(part 1 of 2)
# Autodesk Inventor assembly: #Spindexer
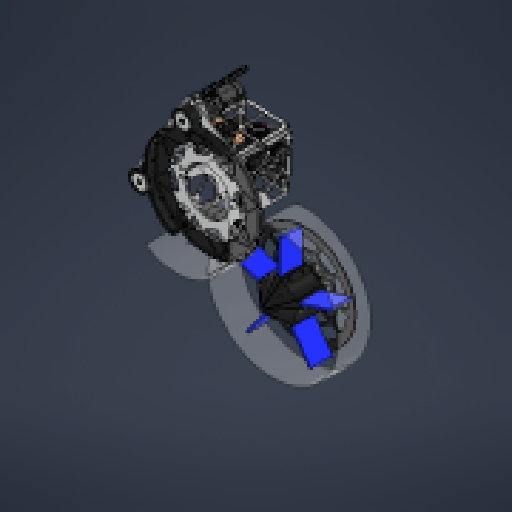
[picture p0: Inventor's stored thumbnail of the model, 512x512]
Saved by Autodesk Inventor 2026.1 (Build 301233020, 233B)
## iProperties
Created: 2026-02-05
Part Number: #Spindexer
Document SubType Name: Assembly
Designer: Owen L
Mass: 7699.55 g
Surface Area: 21817.8 cm^2
Volume: 5845.98 cm^3
Density: 1.31707 g/cm^3
Author: Owen L
## Documents named in this file (69)
- C:\Users\Owen\Documents\GitHub\2026-Robot-Mechanical\Spindexer\#Spindexer.iam
- C:\Users\Owen\Documents\GitHub\2026-Robot-Mechanical\Spindexer\3DPRINT,HUB.ipt
- C:\Users\Owen\Documents\GitHub\2026-Robot-Mechanical\Spindexer\3DPRINT,HUB,CONE.ipt
- C:\Users\Owen\Documents\GitHub\2026-Robot-Mechanical\Spindexer\PLATE,WALL.ipt
- C:\Users\Owen\Documents\GitHub\2026-Robot-Mechanical\Spindexer\PLATE,BOTTOM.ipt
- C:\Users\Owen\Documents\GitHub\2026-Robot-Mechanical\Spindexer\STOCK,HEX,SHAFT,HUB.ipt
- C:\Users\Owen\Documents\GitHub\2026-Robot-Mechanical\Spindexer\PLATE,KICKER,OUTSIDE.ipt
- C:\Users\Owen\Documents\GitHub\2026-Robot-Mechanical\Spindexer\3DPRINT,KICKER,RAMP.ipt
- C:\Users\Owen\Documents\GitHub\2026-Robot-Mechanical\Spindexer\PLATE,KICKER,INSIDE.ipt
- C:\Users\Owen\Documents\GitHub\2026-Robot-Mechanical\Spindexer\STOCK,HEX,SHAFT,KICKER,FRONT.ipt
- C:\Users\Owen\Documents\GitHub\2026-Robot-Mechanical\Spindexer\STOCK,HEX,SHAFT,KICKER,BACK.ipt
- C:\Users\Owen\Documents\GitHub\2026-Robot-Mechanical\#1_CAD Library\Power Transmission\Bearings\PURCHASED,HEX_BEARING.ipt
- C:\Users\Owen\Documents\GitHub\2026-Robot-Mechanical\#1_CAD Library\Power Transmission\VersaPlanetary\GEARBOX,VERSAPLANETARY,SINGLE-STAGE,HEX-SHAFT,0.5IN.ipt
- C:\Users\Owen\Documents\GitHub\2026-Robot-Mechanical\#1_CAD Library\Power Transmission\VersaPlanetary\ADAPTER,CIM-NEO,VERSAPLANETARY.ipt
- C:\Users\Owen\Documents\GitHub\2026-Robot-Mechanical\#1_CAD Library\Motors\MOTOR,REV,NEO,V1-1.ipt
- C:\Users\Owen\Documents\GitHub\2026-Robot-Mechanical\Spindexer\PLATE,NUT-BLOCK,3-LONG.ipt
- C:\Users\Owen\Documents\GitHub\2026-Robot-Mechanical\Spindexer\PLATE,NUT-BLOCK,2-LONG.ipt
- C:\Users\Owen\Documents\GitHub\2026-Robot-Mechanical\Spindexer\PLATE,NUT-BLOCK,1-LONG.ipt
- C:\Users\Owen\Documents\GitHub\2026-Robot-Mechanical\#1_CAD Library\Electronics\CONTROLS,SPARK_MAX.ipt
- C:\Users\Owen\Documents\GitHub\2026-Robot-Mechanical\Spindexer\3DPRINT,SPARK_MAX,MOUNT.ipt
- C:\Users\Owen\Documents\GitHub\2026-Robot-Mechanical\Spindexer\PLATE,KICKER,BACK.ipt
- C:\Users\Owen\Documents\GitHub\2026-Robot-Mechanical\Spindexer\PLATE,NUT-BLOCK,L-SHAPE.ipt
- C:\Users\Owen\Documents\GitHub\2026-Robot-Mechanical\Spindexer\STANDIN,BELT,70T,HTD5mm.ipt
- C:\Users\Owen\Documents\GitHub\2026-Robot-Mechanical\Spindexer\STANDIN,BELT,85T,HTD5mm.ipt
- C:\Users\Owen\Documents\GitHub\2026-Robot-Mechanical\#1_CAD Library\Building Materials\Fasteners\Bolts\PURCHASED,10-32x0.5in,BUTTONHEAD,BOLT.ipt
- C:\Users\Owen\Documents\GitHub\2026-Robot-Mechanical\#1_CAD Library\Building Materials\Fasteners\Nuts\PURCHASED,NYLOCK,10-32,NUT.ipt
- C:\Users\Owen\Documents\GitHub\2026-Robot-Mechanical\#1_CAD Library\Building Materials\Fasteners\Bolts\PURCHASED,10-32x0.625in,BUTTONHEAD,BOLT.ipt
- C:\Users\Owen\Documents\GitHub\2026-Robot-Mechanical\Spindexer\PLATE,NUT-BLOCK,SINGLE-L.ipt
- C:\Users\Owen\Documents\GitHub\2026-Robot-Mechanical\Spindexer\PLATE,SHOOTER,MOUNT.ipt
- C:\Users\Owen\Documents\GitHub\2026-Robot-Mechanical\Spindexer\PLATE,TURRET,ENCODER,GEAR.ipt
- C:\Users\Owen\Documents\GitHub\2026-Robot-Mechanical\Spindexer\PLATE,TURRET,PINNION,GEAR.ipt
- C:\Users\Owen\Documents\GitHub\2026-Robot-Mechanical\Spindexer\PLATE,TURRET,MOTOR,MOUNT.ipt
- C:\Users\Owen\Documents\GitHub\2026-Robot-Mechanical\#1_CAD Library\Electronics\CONTROLS,ENCODER,HEX_BORE.ipt
- C:\Users\Owen\Documents\GitHub\2026-Robot-Mechanical\Spindexer\STOCK,HEX,SHAFT,TURRET,DRIVE.ipt
- C:\Users\Owen\Documents\GitHub\2026-Robot-Mechanical\Spindexer\STOCK,HEX,SHAFT,TURRET,ENCODER.ipt
- C:\Users\Owen\Documents\GitHub\2026-Robot-Mechanical\Spindexer\3DPRINT,TURRET,HEX,SPACER.ipt
- C:\Users\Owen\Documents\GitHub\2026-Robot-Mechanical\Spindexer\STOCK,CHURRO,HEX,TURRET,MOTOR-MOUNT,SPACER.ipt
- C:\Users\Owen\Documents\GitHub\2026-Robot-Mechanical\#1_CAD Library\Building Materials\Fasteners\Bolts\PURCHASED,0.25-20x0.5in,BUTTONHEAD,BOLT.ipt
- C:\Users\Owen\Documents\GitHub\2026-Robot-Mechanical\Spindexer\CAST,SLAB-OF-FLOP.ipt
- C:\Users\Owen\Documents\GitHub\2026-Robot-Mechanical\Spindexer\PURCHASED,20-1,90deg,MAX-PLANETARY.ipt
- C:\Users\Owen\Documents\GitHub\2026-Robot-Mechanical\#1_CAD Library\Motors\MOTOR,NEO,V2.0.ipt
- C:\Users\Owen\Documents\GitHub\2026-Robot-Mechanical\#1_CAD Library\Wheels\Compliant\PURCHASED,WHEEL,COMPLIANT,2.25in.ipt
- C:\Users\Owen\Documents\GitHub\2026-Robot-Mechanical\Spindexer\MOTOR,VEX,FALCON,500.ipt
- C:\Users\Owen\Documents\GitHub\2026-Robot-Mechanical\#1_CAD Library\Power Transmission\MaxPlanetary\PURCHASED,REV,MAX-PLANETARY,SINGLE-STAGE,FALCON-TO-HEX.ipt
- C:\Users\Owen\Documents\GitHub\2026-Robot-Mechanical\#1_CAD Library\Building Materials\Fasteners\Bolts\PURCHASED,10-32x0.625in,FLATHEAD,BOLT.ipt
- C:\Users\Owen\Documents\GitHub\2026-Robot-Mechanical\#1_CAD Library\Building Materials\Fasteners\Washers\PURCHASED,WASHER,10-32.ipt
- C:\Users\Owen\Documents\GitHub\2026-Robot-Mechanical\Spindexer\3DPRINT,21T,HDT5mm,PULLEY.ipt
- C:\Users\Owen\Documents\GitHub\2026-Robot-Mechanical\Spindexer\3DPRINT,24T,HTD5mm,PULLEY.ipt
- C:\Users\Owen\Documents\GitHub\2026-Robot-Mechanical\Spindexer\3DPRINT,KICKER,MOTOR,SPACER.ipt
- C:\Users\Owen\Documents\GitHub\2026-Robot-Mechanical\#1_CAD Library\Power Transmission\Gears\PURCHASED,GEAR,20DP,30T,HEX.ipt
- C:\Users\Owen\Documents\GitHub\2026-Robot-Mechanical\Spindexer\STOCK,HEX,SHAFT,KICKER,REVERSER.ipt
- C:\Users\Owen\Documents\GitHub\2026-Robot-Mechanical\Spindexer\3DPRINT,KICKER,MOTOR,SUPPORT-PLATE,SPACER.ipt
- C:\Users\Owen\Documents\GitHub\2026-Robot-Mechanical\Spindexer\PLATE,KICKER,MOTOR,SUPPORT.ipt
- C:\Users\Owen\Documents\GitHub\2026-Robot-Mechanical\#1_CAD Library\Building Materials\Fasteners\Bolts\PURCHASED,10-32x0.25in,BUTTONHEAD,BOLT.ipt
- C:\Users\Owen\Documents\GitHub\2026-Robot-Mechanical\Spindexer\PLATE,REVERSER,SUPPORT.ipt
- C:\Users\Owen\Documents\GitHub\2026-Robot-Mechanical\Spindexer\STOCK,REVERSER,STANDOFF.ipt
- C:\Users\Owen\Documents\GitHub\2026-Robot-Mechanical\Spindexer\3DPRINT,CABLE-SHROUD,QUARTER.ipt
- C:\Users\Owen\Documents\GitHub\2026-Robot-Mechanical\Spindexer\3DPRINT,CABLE,TRAY,BL.ipt
- C:\Users\Owen\Documents\GitHub\2026-Robot-Mechanical\Spindexer\3DPRINT,CABLE,TRAY,BR.ipt
- C:\Users\Owen\Documents\GitHub\2026-Robot-Mechanical\Spindexer\3DPRINT,CABLE,TRAY,TL.ipt
- C:\Users\Owen\Documents\GitHub\2026-Robot-Mechanical\Spindexer\3DPRINT,CABLE,TRAY,TR.ipt
- C:\Users\Owen\Documents\GitHub\2026-Robot-Mechanical\Spindexer\PLATE,SHOOTER,SHEILD,LOWER.ipt
- C:\Users\Owen\Documents\GitHub\2026-Robot-Mechanical\Spindexer\3DPRINT,TURRET,PINION,SHROUD.ipt
- C:\Users\Owen\Documents\GitHub\2026-Robot-Mechanical\#1_CAD Library\Building Materials\Fasteners\Bolts\PURCHASED,10-32x0.75in,BUTTONHEAD,BOLT.ipt
- C:\Users\Owen\Documents\GitHub\2026-Robot-Mechanical\Spindexer\3DPRINT,TURRET,PINION,SHROUD,21T.ipt
- C:\Users\Owen\Documents\GitHub\2026-Robot-Mechanical\Spindexer\STOCK,CHURRO,HEX,TURRET,MOTOR-MOUNT,SUPPORT.ipt
- C:\Users\Owen\Documents\GitHub\2026-Robot-Mechanical\Spindexer\3DPRINT,TURRET,LOCK.ipt
- C:\Users\Owen\Documents\GitHub\2026-Robot-Mechanical\Spindexer\STOCK,CHURRO,HEX,TURRET,LOCK.ipt
- C:\Users\Owen\Documents\GitHub\2026-Robot-Mechanical\#1_CAD Library\Building Materials\Fasteners\Bolts\PURCHASED,0.25-20x0.875in,SOCKETHEAD,BOLT.ipt
## Components (229 placed, 68 different names)
1. 3DPRINT,TURRET,PINION,SHROUD:1 — Mate:224, Mate:225, Mate:226, Insert:267
2. PURCHASED,10-32x0.75in,BUTTONHEAD,BOLT:1 — Insert:268, Mate:232
3. PURCHASED,10-32x0.75in,BUTTONHEAD,BOLT:2 — Insert:267, Mate:236
4. 3DPRINT,TURRET,PINION,SHROUD,21T:1 — Mate:227, Mate:228, Mate:229, Insert:268
5. STOCK,CHURRO,HEX,TURRET,MOTOR-MOUNT,SPACER:7 — Insert:272
6. STOCK,CHURRO,HEX,TURRET,MOTOR-MOUNT,SPACER:8 — Insert:273
7. PURCHASED,0.25-20x0.5in,BUTTONHEAD,BOLT:16 — Insert:279
8. PURCHASED,0.25-20x0.5in,BUTTONHEAD,BOLT:17 — Insert:280
9. PURCHASED,0.25-20x0.5in,BUTTONHEAD,BOLT:18 — Insert:281
10. STOCK,CHURRO,HEX,TURRET,MOTOR-MOUNT,SUPPORT:1 — Insert:282
11. 3DPRINT,TURRET,LOCK:1 — Mate:237, Mate:238, Flush:35, Insert:285, Insert:286
12. STOCK,CHURRO,HEX,TURRET,LOCK:1 — Insert:283
13. STOCK,CHURRO,HEX,TURRET,LOCK:2 — Insert:284
14. PURCHASED,0.25-20x0.875in,SOCKETHEAD,BOLT:1 — Insert:285
15. PURCHASED,0.25-20x0.875in,SOCKETHEAD,BOLT:2 — Insert:286
16. PURCHASED,0.25-20x0.5in,BUTTONHEAD,BOLT:19 — Insert:287
17. PURCHASED,0.25-20x0.5in,BUTTONHEAD,BOLT:20 — Insert:288
18. PURCHASED,10-32x0.25in,BUTTONHEAD,BOLT:2 — Mate:189, Mate:190
19. PURCHASED,10-32x0.25in,BUTTONHEAD,BOLT:1 — Mate:188, Mate:191
20. PURCHASED,NYLOCK,10-32,NUT:1 — Insert:81
21. PURCHASED,10-32x0.5in,BUTTONHEAD,BOLT:1 — Insert:48
22. PURCHASED,10-32x0.625in,BUTTONHEAD,BOLT:1 — Insert:35
23. PURCHASED,10-32x0.625in,BUTTONHEAD,BOLT:5 — Insert:39
24. PURCHASED,10-32x0.625in,BUTTONHEAD,BOLT:6 — Insert:40
25. PURCHASED,10-32x0.625in,BUTTONHEAD,BOLT:7 — Insert:41
26. PURCHASED,10-32x0.625in,BUTTONHEAD,BOLT:8 — Insert:42
27. PURCHASED,10-32x0.625in,BUTTONHEAD,BOLT:14 — Insert:51
28. PURCHASED,10-32x0.625in,BUTTONHEAD,BOLT:13 — Insert:47
29. PURCHASED,10-32x0.625in,BUTTONHEAD,BOLT:12 — Insert:46
30. PURCHASED,10-32x0.625in,BUTTONHEAD,BOLT:11 — Insert:45
31. PURCHASED,10-32x0.625in,BUTTONHEAD,BOLT:10 — Insert:44
32. PURCHASED,10-32x0.625in,BUTTONHEAD,BOLT:9 — Insert:43
33. PURCHASED,10-32x0.5in,BUTTONHEAD,BOLT:3 — Insert:50
34. PURCHASED,10-32x0.5in,BUTTONHEAD,BOLT:2 — Insert:49
35. PURCHASED,10-32x0.625in,BUTTONHEAD,BOLT:18 — Insert:55
36. PURCHASED,10-32x0.625in,BUTTONHEAD,BOLT:17 — Insert:54
37. PURCHASED,10-32x0.625in,BUTTONHEAD,BOLT:16 — Insert:53
38. PURCHASED,10-32x0.625in,BUTTONHEAD,BOLT:15 — Insert:52
39. PURCHASED,10-32x0.625in,BUTTONHEAD,BOLT:19 — Insert:59
40. PURCHASED,10-32x0.625in,BUTTONHEAD,BOLT:20 — Insert:89
41. PURCHASED,10-32x0.625in,BUTTONHEAD,BOLT:21 — Insert:87
42. PURCHASED,10-32x0.625in,BUTTONHEAD,BOLT:22 — Insert:60
43. PURCHASED,10-32x0.625in,BUTTONHEAD,BOLT:23 — Insert:88
44. PURCHASED,10-32x0.625in,BUTTONHEAD,BOLT:24 — Insert:61
45. PURCHASED,10-32x0.625in,BUTTONHEAD,BOLT:28 — Insert:65
46. PURCHASED,10-32x0.625in,BUTTONHEAD,BOLT:29 — Insert:66
47. PURCHASED,10-32x0.625in,BUTTONHEAD,BOLT:30 — Insert:67
48. PURCHASED,10-32x0.625in,BUTTONHEAD,BOLT:31 — Insert:68
49. PURCHASED,10-32x0.625in,BUTTONHEAD,BOLT:32 — Insert:69
50. PURCHASED,10-32x0.625in,BUTTONHEAD,BOLT:33 — Insert:70
51. PURCHASED,10-32x0.5in,BUTTONHEAD,BOLT:6 — Insert:75
52. PURCHASED,10-32x0.5in,BUTTONHEAD,BOLT:5 — Insert:76
53. PURCHASED,10-32x0.5in,BUTTONHEAD,BOLT:4 — Insert:74
54. PURCHASED,10-32x0.625in,BUTTONHEAD,BOLT:36 — Insert:71
55. PURCHASED,10-32x0.625in,BUTTONHEAD,BOLT:35 — Insert:72
56. PURCHASED,10-32x0.625in,BUTTONHEAD,BOLT:34 — Insert:73
57. PURCHASED,10-32x0.5in,BUTTONHEAD,BOLT:7 — Insert:77
58. PURCHASED,10-32x0.5in,BUTTONHEAD,BOLT:8 — Insert:78
59. PURCHASED,10-32x0.5in,BUTTONHEAD,BOLT:9 — Insert:79
60. PURCHASED,10-32x0.5in,BUTTONHEAD,BOLT:10 — Insert:80
61. PURCHASED,NYLOCK,10-32,NUT:2 — Insert:82
62. PURCHASED,10-32x0.625in,BUTTONHEAD,BOLT:37 — Insert:90
63. PURCHASED,10-32x0.625in,BUTTONHEAD,BOLT:45 — Insert:233
64. PURCHASED,NYLOCK,10-32,NUT:5 — Insert:234
65. PURCHASED,NYLOCK,10-32,NUT:6 — Insert:232
66. PURCHASED,0.25-20x0.5in,BUTTONHEAD,BOLT:9 — Insert:163
67. PURCHASED,0.25-20x0.5in,BUTTONHEAD,BOLT:8 — Insert:162
68. PURCHASED,0.25-20x0.5in,BUTTONHEAD,BOLT:6 — Insert:159
69. PURCHASED,0.25-20x0.5in,BUTTONHEAD,BOLT:5 — Insert:270
70. PURCHASED,NYLOCK,10-32,NUT:8 — Insert:236
71. PURCHASED,NYLOCK,10-32,NUT:7 — Insert:238
72. PURCHASED,10-32x0.625in,BUTTONHEAD,BOLT:47 — Insert:235
73. PURCHASED,0.25-20x0.5in,BUTTONHEAD,BOLT:4 — Insert:158
74. PURCHASED,10-32x0.5in,BUTTONHEAD,BOLT:19 — Insert:247
75. PURCHASED,10-32x0.5in,BUTTONHEAD,BOLT:20 — Insert:248
76. PURCHASED,10-32x0.5in,BUTTONHEAD,BOLT:21 — Insert:249
77. PURCHASED,10-32x0.5in,BUTTONHEAD,BOLT:22 — Insert:250
78. PURCHASED,10-32x0.625in,BUTTONHEAD,BOLT:61 — Insert:174
79. PURCHASED,10-32x0.625in,BUTTONHEAD,BOLT:60 — Insert:175
80. PURCHASED,10-32x0.625in,BUTTONHEAD,BOLT:59 — Insert:176
81. PURCHASED,10-32x0.625in,BUTTONHEAD,BOLT:58 — Insert:177
82. PURCHASED,0.25-20x0.5in,BUTTONHEAD,BOLT:15 — Insert:277
83. PURCHASED,0.25-20x0.5in,BUTTONHEAD,BOLT:14 — Insert:278
84. PURCHASED,0.25-20x0.5in,BUTTONHEAD,BOLT:13
85. PURCHASED,0.25-20x0.5in,BUTTONHEAD,BOLT:12 — Insert:276
86. PURCHASED,0.25-20x0.5in,BUTTONHEAD,BOLT:11 — Insert:169
87. PURCHASED,0.25-20x0.5in,BUTTONHEAD,BOLT:10 — Insert:168
88. PURCHASED,10-32x0.5in,BUTTONHEAD,BOLT:23 — Insert:251
89. PURCHASED,10-32x0.5in,BUTTONHEAD,BOLT:24 — Insert:252
90. PURCHASED,WASHER,10-32:14 — Insert:257
91. PURCHASED,10-32x0.625in,BUTTONHEAD,BOLT:67
92. PURCHASED,WASHER,10-32:15 — Insert:258
93. PURCHASED,10-32x0.625in,BUTTONHEAD,BOLT:68
94. PURCHASED,WASHER,10-32:16 — Insert:259
95. PURCHASED,10-32x0.625in,BUTTONHEAD,BOLT:69
96. PURCHASED,WASHER,10-32:17 — Insert:260
97. PURCHASED,10-32x0.625in,BUTTONHEAD,BOLT:70
98. PURCHASED,WASHER,10-32:18 — Insert:264
99. PURCHASED,10-32x0.625in,BUTTONHEAD,BOLT:71
100. PURCHASED,WASHER,10-32:19 — Insert:263
101. PURCHASED,10-32x0.625in,BUTTONHEAD,BOLT:72
102. PURCHASED,10-32x0.625in,FLATHEAD,BOLT:1 — Insert:185
103. PURCHASED,10-32x0.625in,FLATHEAD,BOLT:2 — Insert:186
104. PURCHASED,10-32x0.625in,FLATHEAD,BOLT:3 — Insert:187
105. PURCHASED,10-32x0.625in,FLATHEAD,BOLT:4 — Insert:188
106. PURCHASED,10-32x0.625in,FLATHEAD,BOLT:5 — Insert:211
107. PURCHASED,10-32x0.625in,FLATHEAD,BOLT:6 — Insert:212
108. PURCHASED,10-32x0.625in,FLATHEAD,BOLT:7 — Insert:214
109. PURCHASED,10-32x0.625in,FLATHEAD,BOLT:8 — Insert:213
110. PURCHASED,WASHER,10-32:11 — Insert:215, Insert:218
111. PURCHASED,WASHER,10-32:12 — Insert:217, Insert:220
112. PURCHASED,WASHER,10-32:13 — Insert:216, Insert:219
113. PURCHASED,10-32x0.625in,BUTTONHEAD,BOLT:62 — Insert:218
114. PURCHASED,10-32x0.625in,BUTTONHEAD,BOLT:63 — Insert:219
115. PURCHASED,10-32x0.625in,BUTTONHEAD,BOLT:64 — Insert:220
116. PURCHASED,10-32x0.5in,BUTTONHEAD,BOLT:11 — Insert:221
117. PURCHASED,10-32x0.5in,BUTTONHEAD,BOLT:13 — Insert:223
118. PURCHASED,10-32x0.5in,BUTTONHEAD,BOLT:12 — Insert:222
119. PURCHASED,10-32x0.5in,BUTTONHEAD,BOLT:14 — Insert:224
120. PURCHASED,10-32x0.5in,BUTTONHEAD,BOLT:15 — Insert:225
121. PURCHASED,10-32x0.5in,BUTTONHEAD,BOLT:16 — Insert:226
122. PURCHASED,10-32x0.5in,BUTTONHEAD,BOLT:17 — Insert:227
123. PURCHASED,10-32x0.5in,BUTTONHEAD,BOLT:18 — Insert:228
124. PURCHASED,10-32x0.625in,BUTTONHEAD,BOLT:65 — Insert:229
125. PURCHASED,10-32x0.625in,BUTTONHEAD,BOLT:66 — Insert:230
126. PURCHASED,10-32x0.625in,FLATHEAD,BOLT:9 — Insert:239
127. PURCHASED,10-32x0.625in,FLATHEAD,BOLT:10 — Insert:240
128. PURCHASED,10-32x0.625in,FLATHEAD,BOLT:11 — Insert:241
129. PURCHASED,10-32x0.625in,FLATHEAD,BOLT:12 — Insert:242
130. PURCHASED,10-32x0.625in,BUTTONHEAD,BOLT:73
131. PURCHASED,WASHER,10-32:20 — Insert:266
132. 3DPRINT,TURRET,HEX,SPACER:1 — Mate:94, Mate:102, Mate:144, Mate:145
133. 3DPRINT,TURRET,HEX,SPACER:2 — Mate:93, Mate:141, Mate:142
134. 3DPRINT,SPARK_MAX,MOUNT:1 — Insert:149, Mate:124, Mate:126, Mate:127
135. 3DPRINT,KICKER,MOTOR,SUPPORT-PLATE,SPACER:1 — Mate:183, Mate:184
136. 3DPRINT,HUB:1 — Mate:11, Mate:12, Mate:13, Mate:15, Mate:16, Mate:17, Flush:2, Mate:106, Mate:107, Mate:108, Mate:109, Mate:110, Mate:111, Mate:112, Mate:113, Mate:114, Mate:117, Mate:118, Mate:119, Mate:120
137. 3DPRINT,HUB,CONE:1 — Mate:11, Mate:12, Mate:13
138. 3DPRINT,KICKER,RAMP:1 — Mate:22, Mate:23, Mate:24
139. 3DPRINT,KICKER,MOTOR,SPACER:1 — Flush:30, Mate:166, Mate:182
140. 3DPRINT,24T,HTD5mm,PULLEY:2 — Mate:161, Mate:182, Mate:184, Mate:193
141. 3DPRINT,24T,HTD5mm,PULLEY:1 — Mate:160, Mate:173, Mate:178
142. 3DPRINT,21T,HDT5mm,PULLEY:2 — Mate:159, Mate:177, Mate:178, Mate:196
143. 3DPRINT,21T,HDT5mm,PULLEY:1 — Mate:164, Mate:180, Mate:181
144. 3DPRINT,CABLE,TRAY,TR:1 — Mate:219, Mate:220
145. 3DPRINT,CABLE,TRAY,TL:1 — Mate:217, Mate:218, Mate:219, Mate:220
146. 3DPRINT,CABLE,TRAY,BR:1 — Mate:215, Mate:216, Mate:217, Mate:218
147. 3DPRINT,CABLE,TRAY,BL:1 — Mate:213, Mate:214, Flush:33, Mate:215, Mate:216
148. 3DPRINT,CABLE-SHROUD,QUARTER:2 — Mate:205, Mate:206, Mate:207, Mate:223, Mate:226
149. 3DPRINT,CABLE-SHROUD,QUARTER:1 — Mate:202, Mate:203, Mate:204, Mate:205, Mate:207, Flush:33, Mate:228
150. PURCHASED,WHEEL,COMPLIANT,2.25in:6 — Mate:132, Mate:135, Mate:139
151. PURCHASED,WHEEL,COMPLIANT,2.25in:5 — Mate:131, Mate:134, Mate:135
152. PURCHASED,WHEEL,COMPLIANT,2.25in:4 — Mate:133, Mate:134
153. PURCHASED,WHEEL,COMPLIANT,2.25in:3 — Mate:130, Mate:136, Mate:138
154. PURCHASED,WHEEL,COMPLIANT,2.25in:2 — Mate:129, Mate:137
155. PURCHASED,WHEEL,COMPLIANT,2.25in:1 — Mate:128, Mate:136, Mate:137
156. CAST,SLAB-OF-FLOP:5 — Mate:114, Mate:120
157. CAST,SLAB-OF-FLOP:4 — Mate:112, Mate:113
158. CAST,SLAB-OF-FLOP:3 — Mate:110, Mate:111
159. CAST,SLAB-OF-FLOP:2 — Mate:108, Mate:109
160. CAST,SLAB-OF-FLOP:1 — Mate:106, Mate:107
161. PLATE,NUT-BLOCK,SINGLE-L:1 — Insert:85, Mate:61
162. PLATE,NUT-BLOCK,SINGLE-L:2 — Insert:86, Mate:62
163. PLATE,NUT-BLOCK,3-LONG:2 — Insert:9, Insert:10
164. PLATE,NUT-BLOCK,3-LONG:3 — Mate:59, Insert:83
165. PLATE,NUT-BLOCK,1-LONG:1 — Insert:13, Flush:11, Flush:12
166. PLATE,NUT-BLOCK,1-LONG:2 — Insert:14, Flush:11
167. PLATE,NUT-BLOCK,3-LONG:4 — Insert:210, Mate:153
168. PLATE,NUT-BLOCK,3-LONG:5 — Insert:93, Insert:94, Mate:152
169. PLATE,NUT-BLOCK,2-LONG:2 — Insert:21, Insert:22, Mate:44, Insert:26
170. PLATE,NUT-BLOCK,2-LONG:3 — Insert:23, Insert:24, Insert:25
171. PLATE,NUT-BLOCK,3-LONG:6 — Insert:27, Insert:28
172. PLATE,NUT-BLOCK,3-LONG:8 — Insert:31, Insert:32
173. PLATE,NUT-BLOCK,L-SHAPE:1 — Insert:33
174. PLATE,NUT-BLOCK,3-LONG:1 — Mate:60, Insert:84
175. PLATE,NUT-BLOCK,L-SHAPE:2 — Insert:34
176. PLATE,KICKER,OUTSIDE:1 — Mate:22, Mate:23, Mate:24, Mate:25, Flush:3, Flush:4, Flush:8, Insert:1, Insert:4, Mate:34, Mate:35, Mate:42, Insert:9, Insert:10, Insert:13, Flush:12, Mate:43, Insert:23, Insert:24, Insert:34, Insert:35, Insert:39, Insert:40, Insert:41, Insert:42, Insert:43, Insert:44, Insert:45, Insert:46, Insert:47, Insert:48, Insert:49, Insert:50, Insert:79, Insert:80, Insert:81, Insert:82, Mate:59, Insert:83, Mate:62, Insert:87, Insert:93, Insert:94, Mate:65, Mate:138, Mate:139, Insert:213, Insert:214
177. PLATE,KICKER,INSIDE:1 — Mate:25, Flush:3, Flush:4, Insert:2, Insert:3, Mate:39, Mate:40, Mate:41, Insert:14, Insert:21, Insert:22, Insert:31, Insert:32, Insert:33, Insert:61, Insert:65, Insert:66, Insert:67, Insert:68, Insert:69, Insert:70, Insert:71, Insert:72, Insert:73, Insert:74, Insert:75, Insert:76, Insert:77, Insert:78, Mate:60, Insert:84, Mate:61, Insert:90, Insert:210, Insert:211, Insert:212, Mate:164, Mate:169, Insert:243, Mate:198, Mate:199, Insert:244, Insert:245, Insert:246, Insert:250, Insert:251, Insert:252
178. PLATE,SHOOTER,MOUNT:1 — Mate:65, Mate:82, Mate:95, Mate:100, Insert:150, Insert:152, Insert:153, Insert:154, Insert:158, Insert:159, Insert:165, Insert:166, Insert:168, Insert:169, Insert:185, Insert:186, Insert:187, Insert:188, Insert:221, Insert:222, Insert:223, Insert:224, Insert:225, Insert:226, Insert:227, Insert:228, Insert:233, Insert:235, Insert:239, Insert:240, Insert:241, Insert:242, Mate:152, Mate:153, Mate:202, Mate:203, Mate:204, Mate:206, Mate:213, Mate:214, Mate:222, Flush:34, Mate:225, Mate:229, Mate:231, Insert:270, Mate:233, Mate:234, Mate:235, Insert:274, Insert:276, Insert:280, Insert:281, Mate:237, Mate:238, Insert:283, Insert:284, Insert:287, Insert:288
179. PLATE,KICKER,BACK:1 — Mate:44, Insert:25, Insert:26, Insert:27, Insert:28, Insert:51, Insert:52, Insert:53, Insert:54, Insert:55, Insert:59, Insert:60, Insert:85, Insert:86, Insert:88, Insert:89, Insert:149, Mate:124, Mate:125, Insert:229, Insert:230
180. PLATE,TURRET,MOTOR,MOUNT:1 — Mate:100, Insert:155, Insert:157, Insert:162, Insert:163, Insert:174, Insert:175, Insert:176, Insert:177, Mate:147, Insert:178, Mate:148, Mate:231, Insert:269, Insert:282
181. PLATE,TURRET,MOTOR,MOUNT:2 — Mate:233, Mate:234, Mate:235, Insert:271, Insert:272, Insert:273, Insert:275, Insert:277, Insert:278, Insert:279
182. PLATE,REVERSER,SUPPORT:1 — Mate:197, Mate:198, Mate:199, Insert:247, Insert:248, Insert:249
183. PLATE,TURRET,ENCODER,GEAR:1 — Mate:102, Mate:143, Flush:26
184. PLATE,TURRET,PINNION,GEAR:1 — Mate:86, Flush:25, Mate:140, Mate:141, Flush:35
185. PLATE,BOTTOM:1 — Mate:117, Mate:118, Mate:119, Flush:24, Mate:122
186. PLATE,KICKER,MOTOR,SUPPORT:1 — Mate:185, Mate:186, Mate:187, Mate:188, Mate:189
187. PLATE,SHOOTER,SHEILD,LOWER:1 — Mate:222, Flush:34, Mate:223
188. PLATE,WALL:1 — Flush:8, Mate:42, Mate:43, Flush:24
189. STOCK,HEX,SHAFT,HUB:1 — Mate:16, Mate:17, Flush:2, Mate:121
190. STOCK,HEX,SHAFT,KICKER,REVERSER:1 — Mate:170, Mate:172, Mate:194, Insert:258, Insert:266
191. STOCK,HEX,SHAFT,KICKER,FRONT:1 — Mate:34, Flush:15, Mate:128, Mate:129, Mate:130, Mate:168, Insert:257, Insert:264
192. STOCK,HEX,SHAFT,KICKER,BACK:1 — Mate:35, Flush:14, Mate:131, Mate:132, Mate:133, Mate:154, Mate:159, Mate:160, Mate:165, Mate:185, Mate:195, Insert:259, Insert:263
193. STOCK,CHURRO,HEX,TURRET,MOTOR-MOUNT,SPACER:5 — Insert:165
194. STOCK,CHURRO,HEX,TURRET,MOTOR-MOUNT,SPACER:6 — Insert:166
195. STOCK,CHURRO,HEX,TURRET,MOTOR-MOUNT,SPACER:4 — Insert:271, Insert:274
196. STOCK,CHURRO,HEX,TURRET,MOTOR-MOUNT,SPACER:3 — Insert:269
197. STOCK,CHURRO,HEX,TURRET,MOTOR-MOUNT,SPACER:2 — Insert:152, Insert:157
198. STOCK,CHURRO,HEX,TURRET,MOTOR-MOUNT,SPACER:1 — Insert:150
199. STOCK,HEX,SHAFT,TURRET,ENCODER:1 — Mate:143, Flush:26, Mate:144, Insert:216, Insert:217, Mate:224
200. STOCK,HEX,SHAFT,TURRET,DRIVE:1 — Flush:25, Mate:140, Mate:142, Insert:215, Mate:227
201. STANDIN,BELT,70T,HTD5mm:1 — Mate:154, Mate:192, Mate:193
202. STANDIN,BELT,85T,HTD5mm:1 — Mate:194, Mate:195, Mate:196
203. GEARBOX,VERSAPLANETARY,SINGLE-STAGE,HEX-SHAFT,0.5IN:1 — Mate:36, Mate:37, Mate:38, Mate:39, Mate:40, Mate:41, Mate:157, Mate:161, Flush:30, Mate:166, Mate:183, Mate:186, Mate:192
204. ADAPTER,CIM-NEO,VERSAPLANETARY:1 — Mate:36, Mate:37, Mate:38, Insert:5
205. MOTOR,REV,NEO,V1-1:1 — Insert:5
206. CONTROLS,SPARK_MAX:1 — Mate:125, Mate:126, Mate:127
207. PURCHASED,HEX_BEARING:6 — Mate:83, Mate:86, Mate:93, Insert:154
208. PURCHASED,HEX_BEARING:7 — Mate:94, Mate:96, Insert:153, Mate:145
209. CONTROLS,ENCODER,HEX_BORE:1 — Mate:95, Mate:96, Insert:236, Insert:238, Mate:236
210. CONTROLS,ENCODER,HEX_BORE:2 — Mate:82, Mate:83, Insert:232, Insert:234, Mate:232
211. PURCHASED,20-1,90deg,MAX-PLANETARY:1 — Mate:121, Mate:122, Insert:148, Mate:123
212. MOTOR,NEO,V2.0:1 — Insert:148, Mate:123
213. PURCHASED,HEX_BEARING:8 — Insert:155
214. MOTOR,VEX,FALCON,500:1 — Insert:179, Mate:149
215. PURCHASED,REV,MAX-PLANETARY,SINGLE-STAGE,FALCON-TO-HEX:1 — Mate:147, Insert:178, Mate:148, Insert:179, Mate:149
216. PURCHASED,HEX_BEARING:1 — Insert:1, Flush:15
217. PURCHASED,HEX_BEARING:2 — Insert:2
218. PURCHASED,HEX_BEARING:3 — Insert:3, Mate:173
219. PURCHASED,HEX_BEARING:4 — Insert:4, Flush:14
220. PURCHASED,HEX_BEARING:13 — Mate:172, Mate:181, Mate:197
221. PURCHASED,HEX_BEARING:12 — Insert:243, Mate:179
222. PURCHASED,GEAR,20DP,30T,HEX:2 — Mate:168, Flush:31
223. PURCHASED,GEAR,20DP,30T,HEX:1 — Mate:169, Flush:31, Mate:170, Mate:179, Mate:180
224. PURCHASED,HEX_BEARING:11 — Mate:165, Flush:29, Mate:177, Mate:191
225. PURCHASED,HEX_BEARING:10 — Mate:157, Flush:29, Mate:187, Mate:190, Insert:260
226. PURCHASED,HEX_BEARING:9 — Insert:275
227. STOCK,REVERSER,STANDOFF:1 — Insert:244
228. STOCK,REVERSER,STANDOFF:2 — Insert:245
229. STOCK,REVERSER,STANDOFF:3 — Insert:246
## Relationships (334: Insert 173, Mate 144, Flush 17)
- Mate:11: 3DPRINT,HUB:1 ↔ 3DPRINT,HUB,CONE:1
- Mate:12: 3DPRINT,HUB:1 ↔ 3DPRINT,HUB,CONE:1
- Mate:13: 3DPRINT,HUB:1 ↔ 3DPRINT,HUB,CONE:1
- Mate:15: 3DPRINT,HUB:1
- Mate:16: 3DPRINT,HUB:1 ↔ STOCK,HEX,SHAFT,HUB:1
- Mate:17: 3DPRINT,HUB:1 ↔ STOCK,HEX,SHAFT,HUB:1
- Flush:2 (-12.7 mm): 3DPRINT,HUB:1 ↔ STOCK,HEX,SHAFT,HUB:1
- Mate:22: 3DPRINT,KICKER,RAMP:1 ↔ PLATE,KICKER,OUTSIDE:1
- Mate:23: 3DPRINT,KICKER,RAMP:1 ↔ PLATE,KICKER,OUTSIDE:1
- Mate:24: 3DPRINT,KICKER,RAMP:1 ↔ PLATE,KICKER,OUTSIDE:1
- Mate:25 (158.75 mm): PLATE,KICKER,OUTSIDE:1 ↔ PLATE,KICKER,INSIDE:1
- Flush:3: PLATE,KICKER,OUTSIDE:1 ↔ PLATE,KICKER,INSIDE:1
- Flush:4: PLATE,KICKER,OUTSIDE:1 ↔ PLATE,KICKER,INSIDE:1
- Flush:8: PLATE,KICKER,OUTSIDE:1 ↔ PLATE,WALL:1
- Insert:1: PLATE,KICKER,OUTSIDE:1 ↔ PURCHASED,HEX_BEARING:1
- Insert:2: PLATE,KICKER,INSIDE:1 ↔ PURCHASED,HEX_BEARING:2
- Insert:3: PLATE,KICKER,INSIDE:1 ↔ PURCHASED,HEX_BEARING:3
- Insert:4: PLATE,KICKER,OUTSIDE:1 ↔ PURCHASED,HEX_BEARING:4
- Mate:34: PLATE,KICKER,OUTSIDE:1 ↔ STOCK,HEX,SHAFT,KICKER,FRONT:1
- Mate:35: PLATE,KICKER,OUTSIDE:1 ↔ STOCK,HEX,SHAFT,KICKER,BACK:1
- Mate:36: GEARBOX,VERSAPLANETARY,SINGLE-STAGE,HEX-SHAFT,0.5IN:1 ↔ ADAPTER,CIM-NEO,VERSAPLANETARY:1
- Mate:37: GEARBOX,VERSAPLANETARY,SINGLE-STAGE,HEX-SHAFT,0.5IN:1 ↔ ADAPTER,CIM-NEO,VERSAPLANETARY:1
- Mate:38: GEARBOX,VERSAPLANETARY,SINGLE-STAGE,HEX-SHAFT,0.5IN:1 ↔ ADAPTER,CIM-NEO,VERSAPLANETARY:1
- Insert:5: ADAPTER,CIM-NEO,VERSAPLANETARY:1 ↔ MOTOR,REV,NEO,V1-1:1
- Mate:39: PLATE,KICKER,INSIDE:1 ↔ GEARBOX,VERSAPLANETARY,SINGLE-STAGE,HEX-SHAFT,0.5IN:1
- Mate:40: PLATE,KICKER,INSIDE:1 ↔ GEARBOX,VERSAPLANETARY,SINGLE-STAGE,HEX-SHAFT,0.5IN:1
- Mate:41: PLATE,KICKER,INSIDE:1 ↔ GEARBOX,VERSAPLANETARY,SINGLE-STAGE,HEX-SHAFT,0.5IN:1
- Mate:42: PLATE,KICKER,OUTSIDE:1 ↔ PLATE,WALL:1
- Insert:9: PLATE,NUT-BLOCK,3-LONG:2 ↔ PLATE,KICKER,OUTSIDE:1
- Insert:10: PLATE,NUT-BLOCK,3-LONG:2 ↔ PLATE,KICKER,OUTSIDE:1
- Insert:13: PLATE,NUT-BLOCK,1-LONG:1 ↔ PLATE,KICKER,OUTSIDE:1
- Insert:14: PLATE,NUT-BLOCK,1-LONG:2 ↔ PLATE,KICKER,INSIDE:1
- Flush:11: PLATE,NUT-BLOCK,1-LONG:1 ↔ PLATE,NUT-BLOCK,1-LONG:2
- Flush:12: PLATE,NUT-BLOCK,1-LONG:1 ↔ PLATE,KICKER,OUTSIDE:1
- Mate:43 (-25.4 mm): PLATE,KICKER,OUTSIDE:1 ↔ PLATE,WALL:1
- Insert:21: PLATE,NUT-BLOCK,2-LONG:2 ↔ PLATE,KICKER,INSIDE:1
- Insert:22: PLATE,NUT-BLOCK,2-LONG:2 ↔ PLATE,KICKER,INSIDE:1
- Insert:23: PLATE,NUT-BLOCK,2-LONG:3 ↔ PLATE,KICKER,OUTSIDE:1
- Insert:24: PLATE,NUT-BLOCK,2-LONG:3 ↔ PLATE,KICKER,OUTSIDE:1
- Mate:44: PLATE,NUT-BLOCK,2-LONG:2 ↔ PLATE,KICKER,BACK:1
- Insert:25: PLATE,NUT-BLOCK,2-LONG:3 ↔ PLATE,KICKER,BACK:1
- Insert:26: PLATE,NUT-BLOCK,2-LONG:2 ↔ PLATE,KICKER,BACK:1
- Insert:27: PLATE,NUT-BLOCK,3-LONG:6 ↔ PLATE,KICKER,BACK:1
- Insert:28: PLATE,NUT-BLOCK,3-LONG:6 ↔ PLATE,KICKER,BACK:1
- Insert:31: PLATE,NUT-BLOCK,3-LONG:8 ↔ PLATE,KICKER,INSIDE:1
- Insert:32: PLATE,NUT-BLOCK,3-LONG:8 ↔ PLATE,KICKER,INSIDE:1
- Insert:33: PLATE,NUT-BLOCK,L-SHAPE:1 ↔ PLATE,KICKER,INSIDE:1
- Insert:34: PLATE,NUT-BLOCK,L-SHAPE:2 ↔ PLATE,KICKER,OUTSIDE:1
- Flush:14: STOCK,HEX,SHAFT,KICKER,BACK:1 ↔ PURCHASED,HEX_BEARING:4
- Flush:15: STOCK,HEX,SHAFT,KICKER,FRONT:1 ↔ PURCHASED,HEX_BEARING:1
- Insert:35: PURCHASED,10-32x0.625in,BUTTONHEAD,BOLT:1 ↔ PLATE,KICKER,OUTSIDE:1
- Insert:39: PURCHASED,10-32x0.625in,BUTTONHEAD,BOLT:5 ↔ PLATE,KICKER,OUTSIDE:1
- Insert:40: PURCHASED,10-32x0.625in,BUTTONHEAD,BOLT:6 ↔ PLATE,KICKER,OUTSIDE:1
- Insert:41: PURCHASED,10-32x0.625in,BUTTONHEAD,BOLT:7 ↔ PLATE,KICKER,OUTSIDE:1
- Insert:42: PURCHASED,10-32x0.625in,BUTTONHEAD,BOLT:8 ↔ PLATE,KICKER,OUTSIDE:1
- Insert:43: PURCHASED,10-32x0.625in,BUTTONHEAD,BOLT:9 ↔ PLATE,KICKER,OUTSIDE:1
- Insert:44: PURCHASED,10-32x0.625in,BUTTONHEAD,BOLT:10 ↔ PLATE,KICKER,OUTSIDE:1
- Insert:45: PURCHASED,10-32x0.625in,BUTTONHEAD,BOLT:11 ↔ PLATE,KICKER,OUTSIDE:1
- Insert:46: PURCHASED,10-32x0.625in,BUTTONHEAD,BOLT:12 ↔ PLATE,KICKER,OUTSIDE:1
- Insert:47: PURCHASED,10-32x0.625in,BUTTONHEAD,BOLT:13 ↔ PLATE,KICKER,OUTSIDE:1
- Insert:48: PURCHASED,10-32x0.5in,BUTTONHEAD,BOLT:1 ↔ PLATE,KICKER,OUTSIDE:1
- Insert:49: PURCHASED,10-32x0.5in,BUTTONHEAD,BOLT:2 ↔ PLATE,KICKER,OUTSIDE:1
- Insert:50: PURCHASED,10-32x0.5in,BUTTONHEAD,BOLT:3 ↔ PLATE,KICKER,OUTSIDE:1
- Insert:51: PURCHASED,10-32x0.625in,BUTTONHEAD,BOLT:14 ↔ PLATE,KICKER,BACK:1
- Insert:52: PURCHASED,10-32x0.625in,BUTTONHEAD,BOLT:15 ↔ PLATE,KICKER,BACK:1
- Insert:53: PURCHASED,10-32x0.625in,BUTTONHEAD,BOLT:16 ↔ PLATE,KICKER,BACK:1
- Insert:54: PURCHASED,10-32x0.625in,BUTTONHEAD,BOLT:17 ↔ PLATE,KICKER,BACK:1
- Insert:55: PURCHASED,10-32x0.625in,BUTTONHEAD,BOLT:18 ↔ PLATE,KICKER,BACK:1
- Insert:59: PURCHASED,10-32x0.625in,BUTTONHEAD,BOLT:19 ↔ PLATE,KICKER,BACK:1
- Insert:60: PURCHASED,10-32x0.625in,BUTTONHEAD,BOLT:22 ↔ PLATE,KICKER,BACK:1
- Insert:61: PURCHASED,10-32x0.625in,BUTTONHEAD,BOLT:24 ↔ PLATE,KICKER,INSIDE:1
- Insert:65: PURCHASED,10-32x0.625in,BUTTONHEAD,BOLT:28 ↔ PLATE,KICKER,INSIDE:1
- Insert:66: PURCHASED,10-32x0.625in,BUTTONHEAD,BOLT:29 ↔ PLATE,KICKER,INSIDE:1
- Insert:67: PURCHASED,10-32x0.625in,BUTTONHEAD,BOLT:30 ↔ PLATE,KICKER,INSIDE:1
- Insert:68: PURCHASED,10-32x0.625in,BUTTONHEAD,BOLT:31 ↔ PLATE,KICKER,INSIDE:1
- Insert:69: PURCHASED,10-32x0.625in,BUTTONHEAD,BOLT:32 ↔ PLATE,KICKER,INSIDE:1
- Insert:70: PURCHASED,10-32x0.625in,BUTTONHEAD,BOLT:33 ↔ PLATE,KICKER,INSIDE:1
- Insert:71: PURCHASED,10-32x0.625in,BUTTONHEAD,BOLT:36 ↔ PLATE,KICKER,INSIDE:1
- Insert:72: PURCHASED,10-32x0.625in,BUTTONHEAD,BOLT:35 ↔ PLATE,KICKER,INSIDE:1
- Insert:73: PURCHASED,10-32x0.625in,BUTTONHEAD,BOLT:34 ↔ PLATE,KICKER,INSIDE:1
- Insert:74: PURCHASED,10-32x0.5in,BUTTONHEAD,BOLT:4 ↔ PLATE,KICKER,INSIDE:1
- Insert:75: PURCHASED,10-32x0.5in,BUTTONHEAD,BOLT:6 ↔ PLATE,KICKER,INSIDE:1
- Insert:76: PURCHASED,10-32x0.5in,BUTTONHEAD,BOLT:5 ↔ PLATE,KICKER,INSIDE:1
- Insert:77: PURCHASED,10-32x0.5in,BUTTONHEAD,BOLT:7 ↔ PLATE,KICKER,INSIDE:1
- Insert:78: PURCHASED,10-32x0.5in,BUTTONHEAD,BOLT:8 ↔ PLATE,KICKER,INSIDE:1
- Insert:79: PURCHASED,10-32x0.5in,BUTTONHEAD,BOLT:9 ↔ PLATE,KICKER,OUTSIDE:1
- Insert:80: PURCHASED,10-32x0.5in,BUTTONHEAD,BOLT:10 ↔ PLATE,KICKER,OUTSIDE:1
- Insert:81: PURCHASED,NYLOCK,10-32,NUT:1 ↔ PLATE,KICKER,OUTSIDE:1
- Insert:82: PURCHASED,NYLOCK,10-32,NUT:2 ↔ PLATE,KICKER,OUTSIDE:1
- Mate:59: PLATE,NUT-BLOCK,3-LONG:3 ↔ PLATE,KICKER,OUTSIDE:1
- Insert:83: PLATE,NUT-BLOCK,3-LONG:3 ↔ PLATE,KICKER,OUTSIDE:1
- Mate:60: PLATE,NUT-BLOCK,3-LONG:1 ↔ PLATE,KICKER,INSIDE:1
- Insert:84: PLATE,NUT-BLOCK,3-LONG:1 ↔ PLATE,KICKER,INSIDE:1
- Insert:85: PLATE,NUT-BLOCK,SINGLE-L:1 ↔ PLATE,KICKER,BACK:1
- Mate:61: PLATE,NUT-BLOCK,SINGLE-L:1 ↔ PLATE,KICKER,INSIDE:1
- Insert:86: PLATE,NUT-BLOCK,SINGLE-L:2 ↔ PLATE,KICKER,BACK:1
- Mate:62: PLATE,NUT-BLOCK,SINGLE-L:2 ↔ PLATE,KICKER,OUTSIDE:1
- Insert:87: PURCHASED,10-32x0.625in,BUTTONHEAD,BOLT:21 ↔ PLATE,KICKER,OUTSIDE:1
- Insert:88: PURCHASED,10-32x0.625in,BUTTONHEAD,BOLT:23 ↔ PLATE,KICKER,BACK:1
- Insert:89: PURCHASED,10-32x0.625in,BUTTONHEAD,BOLT:20 ↔ PLATE,KICKER,BACK:1
- Insert:90: PURCHASED,10-32x0.625in,BUTTONHEAD,BOLT:37 ↔ PLATE,KICKER,INSIDE:1
- Insert:93: PLATE,NUT-BLOCK,3-LONG:5 ↔ PLATE,KICKER,OUTSIDE:1
- Insert:94: PLATE,NUT-BLOCK,3-LONG:5 ↔ PLATE,KICKER,OUTSIDE:1
- Mate:65: PLATE,KICKER,OUTSIDE:1 ↔ PLATE,SHOOTER,MOUNT:1
- Mate:82: PLATE,SHOOTER,MOUNT:1 ↔ CONTROLS,ENCODER,HEX_BORE:2
- Mate:83: PURCHASED,HEX_BEARING:6 ↔ CONTROLS,ENCODER,HEX_BORE:2
- Mate:86: PLATE,TURRET,PINNION,GEAR:1 ↔ PURCHASED,HEX_BEARING:6
- Mate:93: 3DPRINT,TURRET,HEX,SPACER:2 ↔ PURCHASED,HEX_BEARING:6
- Mate:94: 3DPRINT,TURRET,HEX,SPACER:1 ↔ PURCHASED,HEX_BEARING:7
- Mate:95: PLATE,SHOOTER,MOUNT:1 ↔ CONTROLS,ENCODER,HEX_BORE:1
- Mate:96: PURCHASED,HEX_BEARING:7 ↔ CONTROLS,ENCODER,HEX_BORE:1
- Mate:100 (19.05 mm): PLATE,SHOOTER,MOUNT:1 ↔ PLATE,TURRET,MOTOR,MOUNT:1
- Mate:102: 3DPRINT,TURRET,HEX,SPACER:1 ↔ PLATE,TURRET,ENCODER,GEAR:1
- Mate:106: 3DPRINT,HUB:1 ↔ CAST,SLAB-OF-FLOP:1
- Mate:107: 3DPRINT,HUB:1 ↔ CAST,SLAB-OF-FLOP:1
- Mate:108: 3DPRINT,HUB:1 ↔ CAST,SLAB-OF-FLOP:2
- Mate:109: 3DPRINT,HUB:1 ↔ CAST,SLAB-OF-FLOP:2
- Mate:110: 3DPRINT,HUB:1 ↔ CAST,SLAB-OF-FLOP:3
- Mate:111: 3DPRINT,HUB:1 ↔ CAST,SLAB-OF-FLOP:3
- Mate:112: 3DPRINT,HUB:1 ↔ CAST,SLAB-OF-FLOP:4
- Mate:113: 3DPRINT,HUB:1 ↔ CAST,SLAB-OF-FLOP:4
- Mate:114: 3DPRINT,HUB:1 ↔ CAST,SLAB-OF-FLOP:5
- Mate:117: 3DPRINT,HUB:1 ↔ PLATE,BOTTOM:1
- Mate:118: 3DPRINT,HUB:1 ↔ PLATE,BOTTOM:1
- Mate:119: 3DPRINT,HUB:1 ↔ PLATE,BOTTOM:1
- Flush:24 (-3.175 mm): PLATE,BOTTOM:1 ↔ PLATE,WALL:1
- Mate:120: 3DPRINT,HUB:1 ↔ CAST,SLAB-OF-FLOP:5
- Mate:121: STOCK,HEX,SHAFT,HUB:1 ↔ PURCHASED,20-1,90deg,MAX-PLANETARY:1
- Mate:122 (6.35 mm): PLATE,BOTTOM:1 ↔ PURCHASED,20-1,90deg,MAX-PLANETARY:1
- Insert:148: PURCHASED,20-1,90deg,MAX-PLANETARY:1 ↔ MOTOR,NEO,V2.0:1
- Mate:123: PURCHASED,20-1,90deg,MAX-PLANETARY:1 ↔ MOTOR,NEO,V2.0:1
- Insert:149: 3DPRINT,SPARK_MAX,MOUNT:1 ↔ PLATE,KICKER,BACK:1
- Mate:124: 3DPRINT,SPARK_MAX,MOUNT:1 ↔ PLATE,KICKER,BACK:1
- Mate:125: PLATE,KICKER,BACK:1 ↔ CONTROLS,SPARK_MAX:1
- Mate:126: 3DPRINT,SPARK_MAX,MOUNT:1 ↔ CONTROLS,SPARK_MAX:1
- Mate:127: 3DPRINT,SPARK_MAX,MOUNT:1 ↔ CONTROLS,SPARK_MAX:1
- Mate:128: PURCHASED,WHEEL,COMPLIANT,2.25in:1 ↔ STOCK,HEX,SHAFT,KICKER,FRONT:1
- Mate:129: PURCHASED,WHEEL,COMPLIANT,2.25in:2 ↔ STOCK,HEX,SHAFT,KICKER,FRONT:1
- Mate:130: PURCHASED,WHEEL,COMPLIANT,2.25in:3 ↔ STOCK,HEX,SHAFT,KICKER,FRONT:1
- Mate:131: PURCHASED,WHEEL,COMPLIANT,2.25in:5 ↔ STOCK,HEX,SHAFT,KICKER,BACK:1
- Mate:132: PURCHASED,WHEEL,COMPLIANT,2.25in:6 ↔ STOCK,HEX,SHAFT,KICKER,BACK:1
- Mate:133: PURCHASED,WHEEL,COMPLIANT,2.25in:4 ↔ STOCK,HEX,SHAFT,KICKER,BACK:1
- Mate:134: PURCHASED,WHEEL,COMPLIANT,2.25in:5 ↔ PURCHASED,WHEEL,COMPLIANT,2.25in:4
- Mate:135: PURCHASED,WHEEL,COMPLIANT,2.25in:6 ↔ PURCHASED,WHEEL,COMPLIANT,2.25in:5
- Mate:136: PURCHASED,WHEEL,COMPLIANT,2.25in:3 ↔ PURCHASED,WHEEL,COMPLIANT,2.25in:1
- Mate:137: PURCHASED,WHEEL,COMPLIANT,2.25in:2 ↔ PURCHASED,WHEEL,COMPLIANT,2.25in:1
- Mate:138 (41.275 mm): PURCHASED,WHEEL,COMPLIANT,2.25in:3 ↔ PLATE,KICKER,OUTSIDE:1
- Mate:139 (41.275 mm): PURCHASED,WHEEL,COMPLIANT,2.25in:6 ↔ PLATE,KICKER,OUTSIDE:1
- Insert:150: PLATE,SHOOTER,MOUNT:1 ↔ STOCK,CHURRO,HEX,TURRET,MOTOR-MOUNT,SPACER:1
- Insert:152: PLATE,SHOOTER,MOUNT:1 ↔ STOCK,CHURRO,HEX,TURRET,MOTOR-MOUNT,SPACER:2
- Insert:153: PLATE,SHOOTER,MOUNT:1 ↔ PURCHASED,HEX_BEARING:7
- Insert:154: PLATE,SHOOTER,MOUNT:1 ↔ PURCHASED,HEX_BEARING:6
- Insert:155: PLATE,TURRET,MOTOR,MOUNT:1 ↔ PURCHASED,HEX_BEARING:8
- Insert:157: PLATE,TURRET,MOTOR,MOUNT:1 ↔ STOCK,CHURRO,HEX,TURRET,MOTOR-MOUNT,SPACER:2
- Insert:158: PURCHASED,0.25-20x0.5in,BUTTONHEAD,BOLT:4 ↔ PLATE,SHOOTER,MOUNT:1
- Insert:159: PURCHASED,0.25-20x0.5in,BUTTONHEAD,BOLT:6 ↔ PLATE,SHOOTER,MOUNT:1
- Insert:162: PURCHASED,0.25-20x0.5in,BUTTONHEAD,BOLT:8 ↔ PLATE,TURRET,MOTOR,MOUNT:1
- Insert:163: PURCHASED,0.25-20x0.5in,BUTTONHEAD,BOLT:9 ↔ PLATE,TURRET,MOTOR,MOUNT:1
- Flush:25: PLATE,TURRET,PINNION,GEAR:1 ↔ STOCK,HEX,SHAFT,TURRET,DRIVE:1
- Mate:140: PLATE,TURRET,PINNION,GEAR:1 ↔ STOCK,HEX,SHAFT,TURRET,DRIVE:1
- Mate:141: 3DPRINT,TURRET,HEX,SPACER:2 ↔ PLATE,TURRET,PINNION,GEAR:1
- Mate:142: 3DPRINT,TURRET,HEX,SPACER:2 ↔ STOCK,HEX,SHAFT,TURRET,DRIVE:1
- Mate:143: PLATE,TURRET,ENCODER,GEAR:1 ↔ STOCK,HEX,SHAFT,TURRET,ENCODER:1
- Flush:26: PLATE,TURRET,ENCODER,GEAR:1 ↔ STOCK,HEX,SHAFT,TURRET,ENCODER:1
- Mate:144: 3DPRINT,TURRET,HEX,SPACER:1 ↔ STOCK,HEX,SHAFT,TURRET,ENCODER:1
- Mate:145: 3DPRINT,TURRET,HEX,SPACER:1 ↔ PURCHASED,HEX_BEARING:7
- Insert:165: PLATE,SHOOTER,MOUNT:1 ↔ STOCK,CHURRO,HEX,TURRET,MOTOR-MOUNT,SPACER:5
- Insert:166: PLATE,SHOOTER,MOUNT:1 ↔ STOCK,CHURRO,HEX,TURRET,MOTOR-MOUNT,SPACER:6
- Insert:168: PURCHASED,0.25-20x0.5in,BUTTONHEAD,BOLT:10 ↔ PLATE,SHOOTER,MOUNT:1
- Insert:169: PURCHASED,0.25-20x0.5in,BUTTONHEAD,BOLT:11 ↔ PLATE,SHOOTER,MOUNT:1
- Insert:174: PURCHASED,10-32x0.625in,BUTTONHEAD,BOLT:61 ↔ PLATE,TURRET,MOTOR,MOUNT:1
- Insert:175: PURCHASED,10-32x0.625in,BUTTONHEAD,BOLT:60 ↔ PLATE,TURRET,MOTOR,MOUNT:1
- Insert:176: PURCHASED,10-32x0.625in,BUTTONHEAD,BOLT:59 ↔ PLATE,TURRET,MOTOR,MOUNT:1
- Insert:177: PURCHASED,10-32x0.625in,BUTTONHEAD,BOLT:58 ↔ PLATE,TURRET,MOTOR,MOUNT:1
- Mate:147: PLATE,TURRET,MOTOR,MOUNT:1 ↔ PURCHASED,REV,MAX-PLANETARY,SINGLE-STAGE,FALCON-TO-HEX:1
- Insert:178: PLATE,TURRET,MOTOR,MOUNT:1 ↔ PURCHASED,REV,MAX-PLANETARY,SINGLE-STAGE,FALCON-TO-HEX:1
- Mate:148: PLATE,TURRET,MOTOR,MOUNT:1 ↔ PURCHASED,REV,MAX-PLANETARY,SINGLE-STAGE,FALCON-TO-HEX:1
- Insert:179: MOTOR,VEX,FALCON,500:1 ↔ PURCHASED,REV,MAX-PLANETARY,SINGLE-STAGE,FALCON-TO-HEX:1
- Mate:149: MOTOR,VEX,FALCON,500:1 ↔ PURCHASED,REV,MAX-PLANETARY,SINGLE-STAGE,FALCON-TO-HEX:1
- Insert:185: PURCHASED,10-32x0.625in,FLATHEAD,BOLT:1 ↔ PLATE,SHOOTER,MOUNT:1
- Insert:186: PURCHASED,10-32x0.625in,FLATHEAD,BOLT:2 ↔ PLATE,SHOOTER,MOUNT:1
- Insert:187: PURCHASED,10-32x0.625in,FLATHEAD,BOLT:3 ↔ PLATE,SHOOTER,MOUNT:1
- Insert:188: PURCHASED,10-32x0.625in,FLATHEAD,BOLT:4 ↔ PLATE,SHOOTER,MOUNT:1
- Insert:210: PLATE,NUT-BLOCK,3-LONG:4 ↔ PLATE,KICKER,INSIDE:1
- Insert:211: PURCHASED,10-32x0.625in,FLATHEAD,BOLT:5 ↔ PLATE,KICKER,INSIDE:1
- Insert:212: PURCHASED,10-32x0.625in,FLATHEAD,BOLT:6 ↔ PLATE,KICKER,INSIDE:1
- Insert:213: PURCHASED,10-32x0.625in,FLATHEAD,BOLT:8 ↔ PLATE,KICKER,OUTSIDE:1
- Insert:214: PURCHASED,10-32x0.625in,FLATHEAD,BOLT:7 ↔ PLATE,KICKER,OUTSIDE:1
- Insert:215: PURCHASED,WASHER,10-32:11 ↔ STOCK,HEX,SHAFT,TURRET,DRIVE:1
- Insert:216: PURCHASED,WASHER,10-32:13 ↔ STOCK,HEX,SHAFT,TURRET,ENCODER:1
- Insert:217: PURCHASED,WASHER,10-32:12 ↔ STOCK,HEX,SHAFT,TURRET,ENCODER:1
- Insert:218: PURCHASED,WASHER,10-32:11 ↔ PURCHASED,10-32x0.625in,BUTTONHEAD,BOLT:62
- Insert:219: PURCHASED,WASHER,10-32:13 ↔ PURCHASED,10-32x0.625in,BUTTONHEAD,BOLT:63
- Insert:220: PURCHASED,WASHER,10-32:12 ↔ PURCHASED,10-32x0.625in,BUTTONHEAD,BOLT:64
- Insert:221: PURCHASED,10-32x0.5in,BUTTONHEAD,BOLT:11 ↔ PLATE,SHOOTER,MOUNT:1
- Insert:222: PURCHASED,10-32x0.5in,BUTTONHEAD,BOLT:12 ↔ PLATE,SHOOTER,MOUNT:1